# Autodesk Inventor assembly: Omni Roller 8 in
Saved by Autodesk Inventor 2013 (Build 170138000, 138)
## iProperties
Created: 2013-01-07
Part Number: Omni Roller 8 in
Document SubType Name: Assembly
Designer: Nemo
Author: Nemo
## Documents named in this file (4)
- H:\Nemo\Documents\Robotics\VexPro\Wheels\Components\Omni Roller 8 in.iam
- H:\Nemo\Documents\Robotics\VexPro\Omni Wheel\Components\Omni Roller 8 in.ipt
- H:\Nemo\Documents\Robotics\VexPro\Omni Wheel\Components\Omni Roller Shaft 8 in.ipt
- H:\Nemo\Documents\Robotics\VexPro\Omni Wheel\Components\Omni Roller Bearing.ipt
## Components (4 placed, 3 different names)
1. Omni Roller 8 in:1
2. Omni Roller Shaft 8 in:1
3. Omni Roller Bearing:1
4. Omni Roller Bearing:2
## Relationships (4: Mate 2, Insert 2)
- [Mate]: Omni Roller 8 in:1 ↔ Omni Roller Shaft 8 in:1
- [Mate]: Omni Roller 8 in:1 ↔ Omni Roller Shaft 8 in:1
- [Insert]: Omni Roller 8 in:1 ↔ Omni Roller Bearing:1
- [Insert]: Omni Roller 8 in:1 ↔ Omni Roller Bearing:2
